# Autodesk Inventor assembly: montage
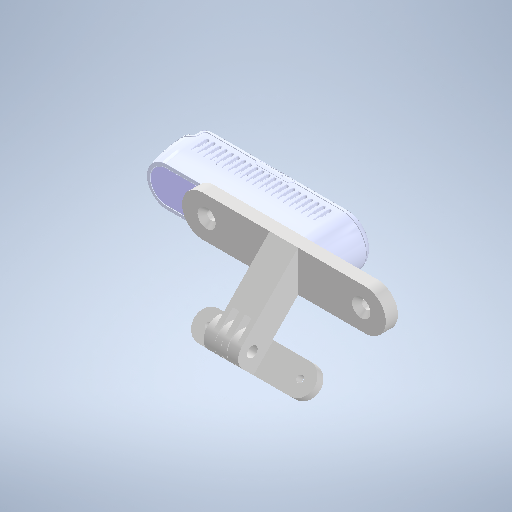
[picture p0: Inventor's stored thumbnail of the model, 512x512]
Saved by Autodesk Inventor 2025.2 (Build 292293000, 293)
## iProperties
Created: 2025-05-12
Part Number: montage
Document SubType Name: Assembly
Designer: enezl
Author: enezl
## Documents named in this file (4)
- E:\Documents\GitHub\CDFR2025\FIPABOT\inventor\realsense\montage.iam
- E:\Documents\GitHub\CDFR2025\FIPABOT\inventor\realsense\support_gopro.ipt
- E:\Documents\GitHub\CDFR2025\FIPABOT\inventor\realsense\support_realsense.ipt
- E:\Documents\ENSTA\CAO_FIPATECH\ROBOT\PINCE\ROBOT\ROBOT\plaque mobile\support_m_v\D435i_Solid\D435i_Solid\D435i_Solid.ipt
## Components (3 placed, 3 different names)
1. support_gopro:1 — Cylindrique:1, Plane:1
2. support_realsense:1 — Cylindrique:1, Plane:1
3. D435i_Solid:1
## Relationships (2: CylindricalJoint 1, PlanarJoint 1)
- Cylindrique:1: support_gopro:1 ↔ support_realsense:1
- Plane:1: support_gopro:1 ↔ support_realsense:1
